# Autodesk Inventor assembly: HERA_NODE_ENCLOSURE_ASSEMBLY
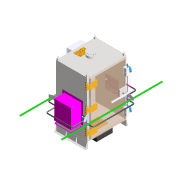
[picture p0: Inventor's stored thumbnail of the model, 180x180]
Saved by Autodesk Inventor 2019.3 (Build 233278000, 278)
## iProperties
Company: ITC Services
Created: 2018-12-14
Part Number: HERA_NODE_ENCLOSURE_ASSEMBLY
Document SubType Name: Assembly
Sending System: Autodesk Inventor 2019
Preprocessor: ST-DEVELOPER v17
Title: D:\ITC\DRAWINGS\SKA PROJECT\HERA NODE\HERA NODE 2018 TENDER SUBMISIONS\ASSEMBLY\HERA_NODE_ENCLOSURE_ASSEMBLY.stp
Author: Francois
Revision Number: 0.2
## Documents named in this file (33)
- C:\Users\Kathryn Rosie\Google Drive\HERA\Node\4. Concept Design\2018-12-14 Post Design Review\HERA_NODE_ENCLOSURE_ASSEMBLY.iam
- C:\Users\Kathryn Rosie\Google Drive\HERA\Node\4. Concept Design\2018-12-14 Post Design Review\HERA_NODE_BOTTOM_PLATE.ipt
- C:\Users\Kathryn Rosie\Google Drive\HERA\Node\4. Concept Design\2018-12-14 Post Design Review\HERA_NODE_LEFT_SIDE_PLATE.ipt
- C:\Users\Kathryn Rosie\Google Drive\HERA\Node\4. Concept Design\2018-12-14 Post Design Review\HERA_NODE_RIGHT_SIDE_PLATE.ipt
- C:\Users\Kathryn Rosie\Google Drive\HERA\Node\4. Concept Design\2018-12-14 Post Design Review\HERA_NODE_TOP_PLATE.ipt
- C:\Users\Kathryn Rosie\Google Drive\HERA\Node\4. Concept Design\2018-12-14 Post Design Review\HERA_NODE_BACK_PLATE.ipt
- C:\Users\Kathryn Rosie\Google Drive\HERA\Node\4. Concept Design\2018-12-14 Post Design Review\HERA_NODE_FOOTPLATE_ASSEMBLY.iam
- C:\Users\Kathryn Rosie\Google Drive\HERA\Node\4. Concept Design\2018-12-14 Post Design Review\HERA_NODE_DOOR_ASSEMBLY.iam
- C:\Users\Kathryn Rosie\Google Drive\HERA\Node\4. Concept Design\2018-12-14 Post Design Review\HINGE_ASSEMBLY.iam
- C:\Users\Kathryn Rosie\Google Drive\HERA\Node\4. Concept Design\2018-12-14 Post Design Review\FILTER_PANEL_COVER_RP.ipt
- C:\Users\Kathryn Rosie\Google Drive\HERA\Node\4. Concept Design\2018-12-14 Post Design Review\LIFTING_LUG_SUPPORT.ipt
- C:\Users\Kathryn Rosie\Google Drive\HERA\Node\4. Concept Design\2018-12-14 Post Design Review\ROOF_PANEL.ipt
- C:\Users\Kathryn Rosie\Google Drive\HERA\Node\4. Concept Design\2018-12-14 Post Design Review\PART 1.ipt
- C:\Users\Kathryn Rosie\Google Drive\HERA\Node\4. Concept Design\2018-12-14 Post Design Review\HERA_NODE_TOP_BOTTOM_ATTENUVENT.ipt
- C:\Users\Kathryn Rosie\Google Drive\HERA\Node\4. Concept Design\2018-12-14 Post Design Review\TS35x7.5 mm H - 6.2 mm dia slot - 225 mm long.ipt
- C:\Users\Kathryn Rosie\Google Drive\HERA\Node\4. Concept Design\2018-12-14 Post Design Review\M10 EYEBOLT.ipt
- C:\Users\Kathryn Rosie\Google Drive\HERA\Node\4. Concept Design\2018-12-14 Post Design Review\FILTER ASSEMBLY.iam
- C:\Users\Kathryn Rosie\Google Drive\HERA\Node\4. Concept Design\2018-12-14 Post Design Review\4-3-4 bullet hinge.ipt
- C:\Users\Kathryn Rosie\Google Drive\HERA\Node\4. Concept Design\2018-12-14 Post Design Review\U_BRACKETS.ipt
- C:\Users\Kathryn Rosie\Google Drive\HERA\Node\4. Concept Design\2018-12-14 Post Design Review\WHIRLEY BIRD.iam
- C:\Users\Kathryn Rosie\Google Drive\HERA\Node\4. Concept Design\2018-12-14 Post Design Review\CABLE_TIE_DOWN_ASSEMBLY.iam
- C:\Users\Kathryn Rosie\Google Drive\HERA\Node\4. Concept Design\2018-12-14 Post Design Review\CARRY_HANDLE_SUPPORT_REV2.ipt
- C:\Users\Kathryn Rosie\Google Drive\HERA\Node\4. Concept Design\2018-12-14 Post Design Review\CARRY_HANDLE_SHORT_REV2.ipt
- C:\Users\Kathryn Rosie\Google Drive\HERA\Node\4. Concept Design\2018-12-14 Post Design Review\CARRY_HANDLE_LONG_REV2.ipt
- C:\Users\Kathryn Rosie\Google Drive\HERA\Node\4. Concept Design\2018-12-14 Post Design Review\DOOR_LOCK_CATCH_REV2.ipt
- C:\Users\Kathryn Rosie\Google Drive\HERA\Node\4. Concept Design\2018-12-14 Post Design Review\TEST LOCKING MECHANISM.iam
- C:\Users\Kathryn Rosie\Google Drive\HERA\Node\4. Concept Design\2018-12-14 Post Design Review\ALBRO_DB_BOX.iam
- C:\Users\Kathryn Rosie\Google Drive\HERA\Node\4. Concept Design\2018-12-14 Post Design Review\Locking pin.iam
- C:\Users\Kathryn Rosie\Google Drive\HERA\Node\4. Concept Design\2018-12-14 Post Design Review\FILTER_PLATE_ASSEMBLY.iam
- C:\Users\Kathryn Rosie\Google Drive\HERA\Node\4. Concept Design\2018-12-14 Post Design Review\FILTER_PLATE_ASSEMBLY_v0.2.iam
- C:\Users\Kathryn Rosie\Google Drive\HERA\Node\4. Concept Design\2018-12-14 Post Design Review\Handle_Bracket.ipt
- C:\Users\Kathryn Rosie\Google Drive\HERA\Node\4. Concept Design\2018-12-14 Post Design Review\Handle_Bracket_Angled.ipt
- C:\Users\Kathryn Rosie\Google Drive\HERA\Node\4. Concept Design\2018-12-14 Post Design Review\Carry_Pole.ipt
## Components (64 placed, 32 different names)
1. HERA_NODE_BOTTOM_PLATE:1 — Flush:3
2. HERA_NODE_LEFT_SIDE_PLATE:1 — Mate:5, Mate:6, Mate:7, Mate:17, Mate:20, Flush:1
3. HERA_NODE_RIGHT_SIDE_PLATE:1 — Mate:2, Mate:3, Mate:4, Mate:14, Mate:23, Mate:24, Flush:1, Mate:27
4. HERA_NODE_TOP_PLATE:1 — Mate:26
5. HERA_NODE_BACK_PLATE:1 — Mate:15, Mate:18, Mate:26, Flush:3, Mate:27
6. HERA_NODE_FOOTPLATE_ASSEMBLY:1 [sub-assembly]
7. HERA_NODE_FOOTPLATE_ASSEMBLY:2 [sub-assembly]
8. HERA_NODE_DOOR_ASSEMBLY:1 [sub-assembly]
9. HINGE_ASSEMBLY:1 [sub-assembly]
10. HINGE_ASSEMBLY:2 [sub-assembly]
11. HINGE_ASSEMBLY:3 [sub-assembly] — Mate:16, Mate:19, Mate:21, Mate:25
12. FILTER_PANEL_COVER_RP:1
13. LIFTING_LUG_SUPPORT:1
14. LIFTING_LUG_SUPPORT:2
15. LIFTING_LUG_SUPPORT:3
16. LIFTING_LUG_SUPPORT:4
17. ROOF_PANEL:1
18. PART 1:1
19. HERA_NODE_TOP_BOTTOM_ATTENUVENT:1
20. HERA_NODE_TOP_BOTTOM_ATTENUVENT:2
21. TS35x7.5 mm H - 6.2 mm dia slot - 225 mm long:1
22. M10 EYEBOLT:1
23. M10 EYEBOLT:2
24. M10 EYEBOLT:3
25. M10 EYEBOLT:4
26. FILTER ASSEMBLY:1 [sub-assembly]
27. 4-3-4 bullet hinge:1
28. 4-3-4 bullet hinge:2
29. U_BRACKETS:2
30. WHIRLEY BIRD:1 [sub-assembly]
31. TS35x7.5 mm H - 6.2 mm dia slot - 225 mm long:2
32. CABLE_TIE_DOWN_ASSEMBLY:1 [sub-assembly]
33. CARRY_HANDLE_SUPPORT_REV2:1
34. CARRY_HANDLE_SUPPORT_REV2:2
35. CARRY_HANDLE_SUPPORT_REV2:3
36. CARRY_HANDLE_SUPPORT_REV2:4
37. CARRY_HANDLE_SHORT_REV2:1
38. CARRY_HANDLE_SHORT_REV2:2
39. CARRY_HANDLE_LONG_REV2:1
40. CARRY_HANDLE_LONG_REV2:2
41. CABLE_TIE_DOWN_ASSEMBLY:2 [sub-assembly]
42. FILTER_PANEL_COVER_RP:2
43. DOOR_LOCK_CATCH_REV2:1
44. DOOR_LOCK_CATCH_REV2:2
45. TEST LOCKING MECHANISM:1 [sub-assembly]
46. ALBRO_DB_BOX:1 [sub-assembly]
47. Locking pin:3 [sub-assembly]
48. Locking pin:4 [sub-assembly]
49. Locking pin:5 [sub-assembly]
50. Locking pin:6 [sub-assembly]
51. Locking pin:7 [sub-assembly]
52. Locking pin:8 [sub-assembly]
53. Locking pin:9 [sub-assembly]
54. Locking pin:10 [sub-assembly]
55. FILTER_PLATE_ASSEMBLY:1 [sub-assembly]
56. FILTER_PLATE_ASSEMBLY:2 [sub-assembly]
57. FILTER_PLATE_ASSEMBLY_v0.2:1 [sub-assembly] — Mate:2, Mate:3, Mate:4
58. FILTER_PLATE_ASSEMBLY_v0.2:2 [sub-assembly] — Mate:5, Mate:6, Mate:7
59. Handle_Bracket:1 — Mate:23, Mate:24, Mate:25, Flush:4, Mate:28
60. Handle_Bracket_Angled:1 — Mate:20, Mate:21
61. Handle_Bracket:3 — Mate:14, Mate:15, Mate:16, Mate:29, Flush:5
62. Handle_Bracket:4 — Mate:17, Mate:18, Mate:19
63. Carry_Pole:1 — Mate:29, Flush:5
64. Carry_Pole:2 — Flush:4, Mate:28
## Relationships (25: Mate 21, Flush 4)
- Mate:2: HERA_NODE_RIGHT_SIDE_PLATE:1 ↔ FILTER_PLATE_ASSEMBLY_v0.2:1
- Mate:3: HERA_NODE_RIGHT_SIDE_PLATE:1 ↔ FILTER_PLATE_ASSEMBLY_v0.2:1
- Mate:4: HERA_NODE_RIGHT_SIDE_PLATE:1 ↔ FILTER_PLATE_ASSEMBLY_v0.2:1
- Mate:5: HERA_NODE_LEFT_SIDE_PLATE:1 ↔ FILTER_PLATE_ASSEMBLY_v0.2:2
- Mate:6: HERA_NODE_LEFT_SIDE_PLATE:1 ↔ FILTER_PLATE_ASSEMBLY_v0.2:2
- Mate:7: HERA_NODE_LEFT_SIDE_PLATE:1 ↔ FILTER_PLATE_ASSEMBLY_v0.2:2
- Mate:14: HERA_NODE_RIGHT_SIDE_PLATE:1 ↔ Handle_Bracket:3
- Mate:15 (-20 mm): HERA_NODE_BACK_PLATE:1 ↔ Handle_Bracket:3
- Mate:16 (5 mm): HINGE_ASSEMBLY:3 ↔ Handle_Bracket:3
- Mate:17: HERA_NODE_LEFT_SIDE_PLATE:1 ↔ Handle_Bracket:4
- Mate:18 (-20 mm): HERA_NODE_BACK_PLATE:1 ↔ Handle_Bracket:4
- Mate:19 (5 mm): HINGE_ASSEMBLY:3 ↔ Handle_Bracket:4
- Mate:20: HERA_NODE_LEFT_SIDE_PLATE:1 ↔ Handle_Bracket_Angled:1
- Mate:21 (5 mm): HINGE_ASSEMBLY:3 ↔ Handle_Bracket_Angled:1
- Mate:23: HERA_NODE_RIGHT_SIDE_PLATE:1 ↔ Handle_Bracket:1
- Mate:24 (-20 mm): HERA_NODE_RIGHT_SIDE_PLATE:1 ↔ Handle_Bracket:1
- Mate:25 (5 mm): HINGE_ASSEMBLY:3 ↔ Handle_Bracket:1
- Flush:1: HERA_NODE_LEFT_SIDE_PLATE:1 ↔ HERA_NODE_RIGHT_SIDE_PLATE:1
- Mate:26: HERA_NODE_TOP_PLATE:1 ↔ HERA_NODE_BACK_PLATE:1
- Flush:3: HERA_NODE_BOTTOM_PLATE:1 ↔ HERA_NODE_BACK_PLATE:1
- Mate:27: HERA_NODE_RIGHT_SIDE_PLATE:1 ↔ HERA_NODE_BACK_PLATE:1
- Flush:4 (-750 mm): Handle_Bracket:1 ↔ Carry_Pole:2
- Mate:28: Handle_Bracket:1 ↔ Carry_Pole:2
- Mate:29: Handle_Bracket:3 ↔ Carry_Pole:1
- Flush:5 (-750 mm): Handle_Bracket:3 ↔ Carry_Pole:1
